# Autodesk Inventor assembly: Motor_v6
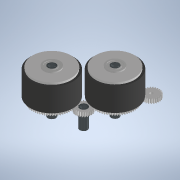
[picture p0: Inventor's stored thumbnail of the model, 180x180]
Saved by Autodesk Inventor 2022 (Build 260153000, 153)
## iProperties
Created: 2022-07-22
Part Number: Motor_v6
Document SubType Name: Assembly
Designer: Yazawa
Author: Yazawa
## Documents named in this file (11)
- C:\Users\Yazawa\Documents\GitHub\murakumo\inventor\Motor_v6.iam
- C:\Users\Yazawa\Documents\GitHub\murakumo\inventor\Tire_v6.iam
- C:\Users\Yazawa\Documents\GitHub\murakumo\inventor\MotorBracket_v6.ipt
- C:\Users\Yazawa\Documents\GitHub\murakumo\inventor\maxon DCX 10L.iam
- C:\Users\Yazawa\Documents\GitHub\murakumo\inventor\FL674ZZ.ipt
- C:\Users\Yazawa\Documents\GitHub\murakumo\inventor\shaft_short.ipt
- C:\Users\Yazawa\Documents\GitHub\murakumo\inventor\pinion_middle_25.ipt
- C:\Users\Yazawa\Documents\GitHub\murakumo\inventor\pinion_source_25.ipt
- C:\Users\Yazawa\Documents\GitHub\murakumo\inventor\Motor_v6\デザイン アクセラレータ\平歯車4.iam
- C:\Users\Yazawa\Documents\GitHub\murakumo\inventor\Motor_v6\デザイン アクセラレータ\平歯車5.iam
- C:\Users\Yazawa\Documents\GitHub\murakumo\inventor\Motor_v6\デザイン アクセラレータ\平歯車6.iam
## Components (12 placed, 8 different names)
1. Tire_v6:1 [sub-assembly] — メイト:5, フラッシュ:2, フラッシュ:5, 正接:1, 正接:2, 正接:5, 正接:6
2. Tire_v6:2 [sub-assembly] — メイト:4, フラッシュ:1, フラッシュ:4, 正接:3, 正接:4
3. MotorBracket_v6:1 — メイト:1, メイト:2, メイト:3, メイト:4, メイト:5, メイト:6, メイト:7, メイト:8, フラッシュ:1, フラッシュ:2, メイト:12, メイト:13
4. maxon DCX 10L:1 [sub-assembly] — メイト:1, メイト:2, メイト:3, メイト:9
5. FL674ZZ:1 — メイト:6, メイト:7, メイト:8, メイト:11
6. shaft_short:1 — メイト:10, メイト:11, フラッシュ:3
7. pinion_middle_25:1 — メイト:10, フラッシュ:3, フラッシュ:4, 正接:2, 正接:3, 正接:4, 正接:5
8. pinion_source_25:1 — メイト:9, フラッシュ:5, 正接:1, 正接:6
9. FL674ZZ:2 — メイト:12, メイト:13
10. 平歯車:1 [sub-assembly]
11. 平歯車:2 [sub-assembly]
12. 平歯車:3 [sub-assembly]
## Relationships (24: Mate 13, Tangent 6, Flush 5)
- メイト:1 [Mate]: MotorBracket_v6:1 ↔ maxon DCX 10L:1
- メイト:2 [Mate]: MotorBracket_v6:1 ↔ maxon DCX 10L:1
- メイト:3 [Mate]: MotorBracket_v6:1 ↔ maxon DCX 10L:1
- メイト:4 [Mate]: Tire_v6:2 ↔ MotorBracket_v6:1
- メイト:5 [Mate]: Tire_v6:1 ↔ MotorBracket_v6:1
- メイト:6 [Mate]: MotorBracket_v6:1 ↔ FL674ZZ:1
- メイト:7 [Mate]: MotorBracket_v6:1 ↔ FL674ZZ:1
- メイト:8 [Mate]: MotorBracket_v6:1 ↔ FL674ZZ:1
- フラッシュ:1 [Flush]: Tire_v6:2 ↔ MotorBracket_v6:1
- フラッシュ:2 [Flush]: Tire_v6:1 ↔ MotorBracket_v6:1
- メイト:9 [Mate]: maxon DCX 10L:1 ↔ pinion_source_25:1
- メイト:10 [Mate]: shaft_short:1 ↔ pinion_middle_25:1
- メイト:11 [Mate]: FL674ZZ:1 ↔ shaft_short:1
- フラッシュ:3 [Flush]: shaft_short:1 ↔ pinion_middle_25:1
- フラッシュ:4 [Flush]: Tire_v6:2 ↔ pinion_middle_25:1
- フラッシュ:5 [Flush]: Tire_v6:1 ↔ pinion_source_25:1
- 正接:1 [Tangent]: Tire_v6:1 ↔ pinion_source_25:1
- 正接:2 [Tangent]: Tire_v6:1 ↔ pinion_middle_25:1
- 正接:3 [Tangent]: Tire_v6:2 ↔ pinion_middle_25:1
- メイト:12 [Mate]: MotorBracket_v6:1 ↔ FL674ZZ:2
- メイト:13 [Mate]: MotorBracket_v6:1 ↔ FL674ZZ:2
- 正接:4 [Tangent]: Tire_v6:2 ↔ pinion_middle_25:1
- 正接:5 [Tangent]: Tire_v6:1 ↔ pinion_middle_25:1
- 正接:6 [Tangent]: Tire_v6:1 ↔ pinion_source_25:1
